# Autodesk Inventor assembly: håndfang bund
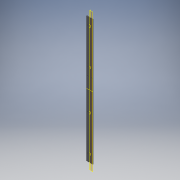
[picture p0: Inventor's stored thumbnail of the model, 180x180]
Saved by Autodesk Inventor 2018 (Build 220112000, 112)
## iProperties
Created: 2019-09-28
Part Number: håndfang bund
Document SubType Name: Assembly
Designer: loppen
Mass: 2394.55 g
Surface Area: 1481.85 cm^2
Volume: 305.039 cm^3
Density: 7.85 g/cm^3
Author: loppen
## Documents named in this file (3)
- Z:\trappe\håndfang\håndfang bund.iam
- Z:\trappe\håndfang\håndfang.ipt
- Z:\trappe\håndfang\afstandsstykke kort.ipt
## Components (6 placed, 2 different names)
1. håndfang:1 — Flush:1, Flush:2, Mate:1, Symmetry:1
2. håndfang:2 — Flush:1, Flush:2, Mate:1, Symmetry:1, Flush:3, Flush:5, Flush:6, Flush:7, Flush:8, Mate:4, Mate:5, Mate:6, Mate:7, Flush:9
3. afstandsstykke kort:1 — Flush:8, Mate:7, Flush:9, Mate:9
4. afstandsstykke kort:2 — Flush:7, Mate:6, Mate:9
5. afstandsstykke kort:3 — Flush:6, Mate:5, Mate:10
6. afstandsstykke kort:4 — Flush:5, Mate:4, Mate:10
## Relationships (16: Flush 8, Mate 7, Symmetry 1)
- Flush:1: håndfang:1 ↔ håndfang:2
- Flush:2: håndfang:1 ↔ håndfang:2
- Mate:1 (-60 mm): håndfang:1 ↔ håndfang:2
- Symmetry:1: håndfang:1 ↔ håndfang:2
- Flush:3: håndfang:2
- Flush:5: håndfang:2 ↔ afstandsstykke kort:4
- Flush:6: håndfang:2 ↔ afstandsstykke kort:3
- Flush:7: håndfang:2 ↔ afstandsstykke kort:2
- Flush:8: håndfang:2 ↔ afstandsstykke kort:1
- Mate:4: håndfang:2 ↔ afstandsstykke kort:4
- Mate:5: håndfang:2 ↔ afstandsstykke kort:3
- Mate:6: håndfang:2 ↔ afstandsstykke kort:2
- Mate:7: håndfang:2 ↔ afstandsstykke kort:1
- Flush:9 (-60 mm): håndfang:2 ↔ afstandsstykke kort:1
- Mate:9 (326.317 mm): afstandsstykke kort:1 ↔ afstandsstykke kort:2
- Mate:10 (326.317 mm): afstandsstykke kort:3 ↔ afstandsstykke kort:4
